# Autodesk Inventor assembly: manipulator
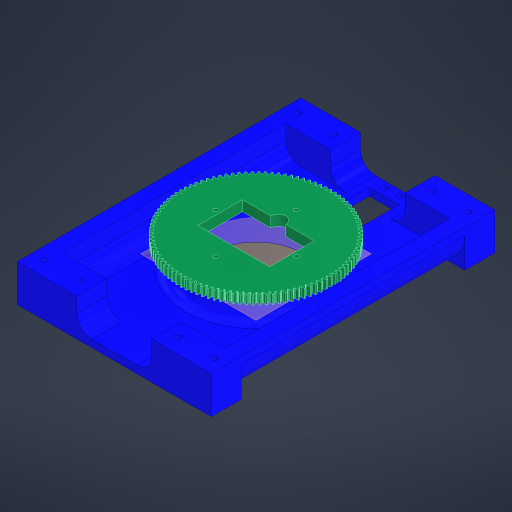
[picture p0: Inventor's stored thumbnail of the model, 512x512]
Saved by Autodesk Inventor 2024 (Build 280153000, 153)
## iProperties
Created: 2023-11-07
Part Number: manipulator
Document SubType Name: Assembly
Designer: user
Author: user
## Documents named in this file (4)
- D:\Docs\Robot\3d_v2\machine_body\manipulator.iam
- D:\Docs\Robot\3d_v2\machine_body\manipulator\platform.ipt
- D:\Docs\Robot\3d_v2\machine_body\manipulator\ring.ipt
- D:\Docs\Robot\3d_v2\machine_body\manipulator\driven_gear.ipt
## Components (3 placed, 3 different names)
1. platform:2 — Совмещение:1, Совмещение:2, Совмещение:3, Заподлицо:1, Заподлицо:2
2. ring:1 — Заподлицо:1, Заподлицо:2, Вставка:1
3. driven_gear:1 — Вставка:1
## Relationships (6: Mate 3, Flush 2, Insert 1)
- Совмещение:1 [Mate]: platform:2
- Совмещение:2 [Mate]: platform:2
- Совмещение:3 [Mate]: platform:2
- Заподлицо:1 [Flush]: platform:2 ↔ ring:1
- Заподлицо:2 [Flush]: platform:2 ↔ ring:1
- Вставка:1 [Insert]: ring:1 ↔ driven_gear:1
